# Autodesk Inventor assembly: SmarDrill
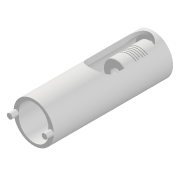
[picture p0: Inventor's stored thumbnail of the model, 180x180]
Saved by Autodesk Inventor 2020 (Build 240168000, 168)
## iProperties
Created: 2020-08-21
Part Number: SmarDrill
Document SubType Name: Assembly
Designer: Jhyatt
Author: Jhyatt
## Documents named in this file (3)
- G:\My Drive\Research Content\Induction Forming\Aluminum Slumping\Engineering\Smart Drill\SmarDrill.iam
- G:\My Drive\Research Content\Induction Forming\Aluminum Slumping\Engineering\Smart Drill\Lock.ipt
- G:\My Drive\Research Content\Induction Forming\Aluminum Slumping\Engineering\Smart Drill\9861T532_ALUMINUM HELICAL FLEXIBLE SHAFT COUPLING.ipt
## Components (2 placed, 2 different names)
1. Lock:1 — Insert:1
2. 9861T532_ALUMINUM HELICAL FLEXIBLE SHAFT COUPLING:1 — Insert:1
## Relationships (1: Insert 1)
- Insert:1: Lock:1 ↔ 9861T532_ALUMINUM HELICAL FLEXIBLE SHAFT COUPLING:1
